# Autodesk Inventor assembly: UNLHEP-14-A-01-006_Rubberstamp
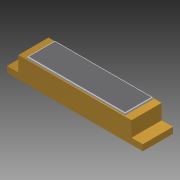
[picture p0: Inventor's stored thumbnail of the model, 180x180]
Saved by Autodesk Inventor 2013 (Build 170138000, 138)
## iProperties
Created: 2014-01-23
Part Number: UNLHEP-14-A-01-006_Rubberstamp
Document SubType Name: Assembly
Designer: Frank Meier
Project: UNL Pixel Phase I
Author: Frank Meier
## Documents named in this file (3)
- C:\Users\Frank Meier\Documents\Inventor\Delvotec-Saugplatte\UNLHEP-14-01-A-006_Rubberstamp.iam
- C:\Users\Frank Meier\Documents\Inventor\Delvotec-Saugplatte\UNLHEP-14-01-P-012_StampPlate.ipt
- C:\Users\Frank Meier\Documents\Inventor\Delvotec-Saugplatte\UNLHEP-14-01-P-011_Rubberstamp.ipt
## Components (2 placed, 2 different names)
1. UNLHEP-14-01-P-012_StampPlate:1 — Passend:1, Passend:2, Passend:3
2. UNLHEP-14-01-P-011_Rubberstamp:1 — Passend:1, Passend:2, Passend:3
## Relationships (3: Mate 3)
- Passend:1 [Mate]: UNLHEP-14-01-P-012_StampPlate:1 ↔ UNLHEP-14-01-P-011_Rubberstamp:1
- Passend:2 [Mate] (-5 mm): UNLHEP-14-01-P-012_StampPlate:1 ↔ UNLHEP-14-01-P-011_Rubberstamp:1
- Passend:3 [Mate] (0.75 mm): UNLHEP-14-01-P-012_StampPlate:1 ↔ UNLHEP-14-01-P-011_Rubberstamp:1
